# Autodesk Inventor assembly: low_shaft
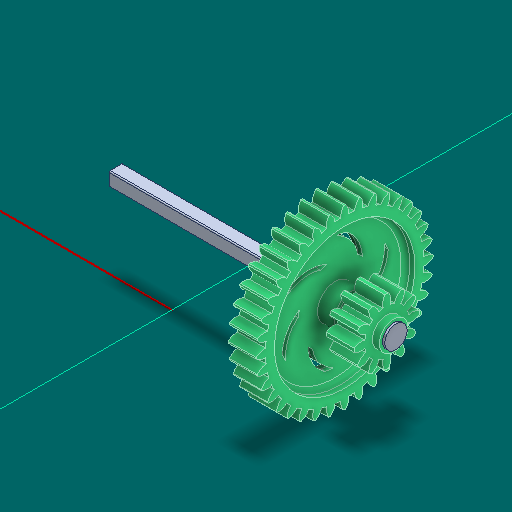
[picture p0: Inventor's stored thumbnail of the model, 512x512]
Saved by Autodesk Inventor 2025 (Build 290162000, 162)
## iProperties
Created: 2024-08-16
Part Number: low_shaft
Document SubType Name: Assembly
Designer: averey
Author: averey
## Documents named in this file (7)
- C:\Users\avere\vex_robotics_high_stakes\hardware\cad\ATLAS\chassis\drive_pod\gearbox\low_shaft.iam
- C:\Users\avere\vex_robotics_high_stakes\hardware\cad\VEX-CAD-Inventor\Motion\Shaft LS\Shaft LS Capped\Shaft LS Capped 2.5.ipt
- C:\Users\avere\vex_robotics_high_stakes\hardware\cad\VEX-CAD-Inventor\Motion\Shaft LS\Shaft LS Capped.ipt
- C:\Users\avere\vex_robotics_high_stakes\hardware\cad\VEX-CAD-Inventor\Motion\Gears\LS 12T Gear.ipt
- C:\Users\avere\vex_robotics_high_stakes\hardware\cad\VEX-CAD-Inventor\Motion\Gears\LS 36T Gear.ipt
- C:\Users\avere\vex_robotics_high_stakes\hardware\cad\VEX-CAD-Inventor\Motion\Spacers\Washer Steel\SWasher .375 OD x .015625.ipt
- C:\Users\avere\vex_robotics_high_stakes\hardware\cad\VEX-CAD-Inventor\Motion\Spacers\Washer Steel.ipt
## Components (4 placed, 4 different names)
1. Shaft LS Capped 2.5:1 — Insert:1, Angle:1, Angle:2
2. LS 12T Gear:1 — Insert:1, Insert:2, Angle:2
3. LS 36T Gear:1 — Insert:2, Insert:3, Angle:1
4. SWasher .375 OD x .015625:1 — Insert:3
## Relationships (5: Insert 3, Angle 2)
- Insert:1: Shaft LS Capped 2.5:1 ↔ LS 12T Gear:1
- Insert:2: LS 12T Gear:1 ↔ LS 36T Gear:1
- Insert:3: LS 36T Gear:1 ↔ SWasher .375 OD x .015625:1
- Angle:1 (0 deg): Shaft LS Capped 2.5:1 ↔ LS 36T Gear:1
- Angle:2 (0 deg): Shaft LS Capped 2.5:1 ↔ LS 12T Gear:1
